# Autodesk Inventor assembly: LOC00011
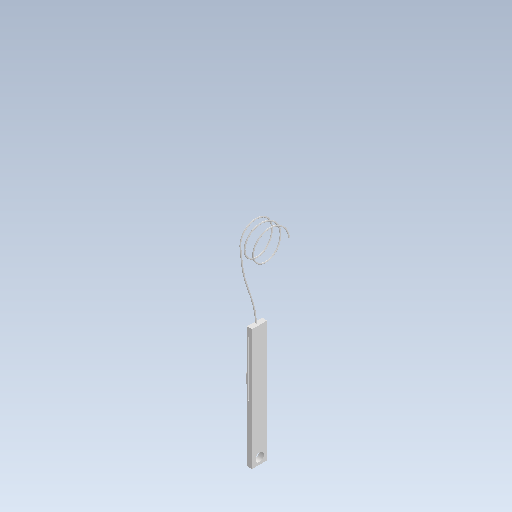
[picture p0: Inventor's stored thumbnail of the model, 512x512]
Saved by Autodesk Inventor 2020 (Build 240168000, 168)
## iProperties
Created: 2021-01-30
Part Number: LOC00011
Document SubType Name: Assembly
Designer: kishore.balu
Description: Caliper System
Engineer: LOKESH BABU/SRI SAI
Author: kishore.balu
Title: MABC-N
Revision Number: 00
## Documents named in this file (5)
- C:\Users\kishore.balu\Documents\LK\New folder\New folder\Caliper-asembly.iam
- C:\Users\kishore.balu\Documents\LK\New folder\New folder\scissor.prt.ipt
- C:\Users\kishore.balu\Documents\LK\New folder\shoes.prt.ipt
- C:\Users\kishore.balu\Documents\LK\New folder\New folder\Thread.ipt
- C:\Users\kishore.balu\Documents\LK\New folder\New folder\Spring.ipt
## Components (4 placed, 4 different names)
1. scissor.prt:1 — Mate:1, Mate:2, Mate:5
2. shoes.prt:1 — Mate:1, Mate:2, Mate:3, Mate:4, Mate:5, Mate:7
3. Thread:1 — Mate:3, Mate:4, Mate:6
4. Spring:1 — Mate:6, Mate:7
## Relationships (7: Mate 7)
- Mate:1: scissor.prt:1 ↔ shoes.prt:1
- Mate:2 (10 mm): scissor.prt:1 ↔ shoes.prt:1
- Mate:3: shoes.prt:1 ↔ Thread:1
- Mate:4: shoes.prt:1 ↔ Thread:1
- Mate:5: scissor.prt:1 ↔ shoes.prt:1
- Mate:6: Thread:1 ↔ Spring:1
- Mate:7: shoes.prt:1 ↔ Spring:1
